# Autodesk Inventor assembly: ENSAMBLE PUERTA M 2021-4.5L
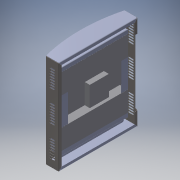
[picture p0: Inventor's stored thumbnail of the model, 180x180]
Saved by Autodesk Inventor 2017 (Build 210142000, 142)
## iProperties
Created: 2021-03-24
Part Number: ENSAMBLE PUERTA M 2021-4.5L
Document SubType Name: Assembly
Designer: USUARIO
Author: USUARIO
Revision Number: ANY
## Documents named in this file (7)
- D:\Laboratorio\Mufla\2021\Mufla 4.5L Psoc MYC Lab #0045885XX OP202145\Modelo\ENSAMBLE PUERTA M 2021-4.5L.iam
- D:\Laboratorio\Mufla\2021\Mufla 4.5L Psoc MYC Lab #0045885XX OP202145\Modelo\ENSAMBLE CUERPO PUERTA M 2021-4.5L.iam
- D:\Laboratorio\Mufla\2021\Mufla 4.5L Psoc MYC Lab #0045885XX OP202145\Modelo\CONTRATAPA EXTERIOR M 2021-4.5L.ipt
- D:\Laboratorio\Mufla\2021\Mufla 4.5L Psoc MYC Lab #0045885XX OP202145\Modelo\CONTRATAPA INTERIOR M 2021-4.5L.ipt
- D:\Laboratorio\Mufla\2021\Mufla 4.5L Psoc MYC Lab #0045885XX OP202145\Modelo\PiezaPuerta-1.ipt
- D:\Laboratorio\Mufla\2021\Mufla 4.5L Psoc MYC Lab #0045885XX OP202145\Modelo\PiezaPuerta-2.ipt
- D:\Laboratorio\Mufla\2021\Mufla 4.5L Psoc MYC Lab #0045885XX OP202145\Modelo\PiezaPuerta-3.ipt
## Components (9 placed, 6 different names)
1. ENSAMBLE CUERPO PUERTA M 2021-4.5L_21 [sub-assembly]
2. CONTRATAPA EXTERIOR M 2021-4.5L_22
3. CONTRATAPA INTERIOR M 2021-4.5L_23 — Mate:1, Mate:2, Mate:3, Mate:4, Mate:5, Mate:6, Mate:7, Mate:8, Mate:9, Mate:11, Mate:12, Mate:18, Mate:19
4. PiezaPuerta-1:1 — Mate:1, Mate:2, Mate:5, Mate:13
5. PiezaPuerta-2:1 — Mate:3, Mate:4, Mate:10
6. PiezaPuerta-1:2 — Mate:6, Mate:7, Mate:21
7. PiezaPuerta-2:2 — Mate:8, Mate:9, Mate:10, Mate:20
8. PiezaPuerta-1:3 — Mate:11, Mate:12, Mate:13
9. PiezaPuerta-3:1 — Mate:18, Mate:19, Mate:20, Mate:21
## Relationships (17: Mate 17)
- Mate:1: CONTRATAPA INTERIOR M 2021-4.5L_23 ↔ PiezaPuerta-1:1
- Mate:2: CONTRATAPA INTERIOR M 2021-4.5L_23 ↔ PiezaPuerta-1:1
- Mate:3: CONTRATAPA INTERIOR M 2021-4.5L_23 ↔ PiezaPuerta-2:1
- Mate:4: CONTRATAPA INTERIOR M 2021-4.5L_23 ↔ PiezaPuerta-2:1
- Mate:5 (1 mm): CONTRATAPA INTERIOR M 2021-4.5L_23 ↔ PiezaPuerta-1:1
- Mate:6: CONTRATAPA INTERIOR M 2021-4.5L_23 ↔ PiezaPuerta-1:2
- Mate:7: CONTRATAPA INTERIOR M 2021-4.5L_23 ↔ PiezaPuerta-1:2
- Mate:8: CONTRATAPA INTERIOR M 2021-4.5L_23 ↔ PiezaPuerta-2:2
- Mate:9: CONTRATAPA INTERIOR M 2021-4.5L_23 ↔ PiezaPuerta-2:2
- Mate:10: PiezaPuerta-2:1 ↔ PiezaPuerta-2:2
- Mate:11: CONTRATAPA INTERIOR M 2021-4.5L_23 ↔ PiezaPuerta-1:3
- Mate:12: CONTRATAPA INTERIOR M 2021-4.5L_23 ↔ PiezaPuerta-1:3
- Mate:13: PiezaPuerta-1:1 ↔ PiezaPuerta-1:3
- Mate:18: CONTRATAPA INTERIOR M 2021-4.5L_23 ↔ PiezaPuerta-3:1
- Mate:19: CONTRATAPA INTERIOR M 2021-4.5L_23 ↔ PiezaPuerta-3:1
- Mate:20: PiezaPuerta-2:2 ↔ PiezaPuerta-3:1
- Mate:21: PiezaPuerta-1:2 ↔ PiezaPuerta-3:1
